# Autodesk Inventor assembly: AxleAssembly
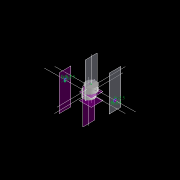
[picture p0: Inventor's stored thumbnail of the model, 180x180]
Saved by Autodesk Inventor 2022.2 (Build 262287010, 287A)
## iProperties
Created: 2022-06-08
Part Number: AxleAssembly
Document SubType Name: Assembly
Designer: Árni Þór Þorgeirsson
Author: Árni Þór Þorgeirsson
## Documents named in this file (3)
- G:\My Drive\Masters Thesis - exo\CAD_Files\ExoskeletonV0p2\Axl\AxleAssembly.iam
- G:\My Drive\Masters Thesis - exo\CAD_Files\ExoskeletonV0p2\Rotor_TSB\PrintingTests\Axle_Printing_TestsRotor_TSB.ipt
- G:\My Drive\Masters Thesis - exo\CAD_Files\ExoskeletonV0p2\Rotor_TSB\PrintingTests\Axle2_Printing_TestsRotor_TSB.ipt
## Components (2 placed, 2 different names)
1. Axle_Printing_TestsRotor_TSB:1 — Insert:1, Insert:2
2. Axle2_Printing_TestsRotor_TSB:1 — Insert:1, Insert:2
## Relationships (2: Insert 2)
- Insert:1: Axle_Printing_TestsRotor_TSB:1 ↔ Axle2_Printing_TestsRotor_TSB:1
- Insert:2: Axle_Printing_TestsRotor_TSB:1 ↔ Axle2_Printing_TestsRotor_TSB:1
